# Autodesk Inventor assembly: Carcasa
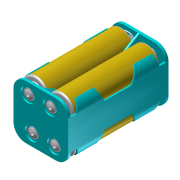
[picture p0: Inventor's stored thumbnail of the model, 180x180]
Saved by Autodesk Inventor 2013 (Build 170138000, 138)
## iProperties
Created: 2015-06-07
Part Number: Carcasa
Document SubType Name: Assembly
Designer: Luis
Author: Luis
## Documents named in this file (3)
- C:\Users\Luis\Documents\Inventor\Bateria\Carcasa.iam
- C:\Users\Luis\Documents\Inventor\Bateria\Imported Components\AABattery Holder\AABattery Holder.ipt
- C:\Users\Luis\Documents\Inventor\Bateria\Imported Components\battery-aa_1-5v\battery-aa_1-5v.ipt
## Components (6 placed, 2 different names)
1. AABattery Holder:1 — Mate:1, Flush:1, Flush:2, Tangent:1, Tangent:2, Mate:2, Tangent:3, Tangent:4, Mate:3
2. AABattery Holder:2 — Mate:1, Flush:1, Flush:2, Tangent:5, Tangent:6, Tangent:7, Tangent:8, Mate:4, Mate:5
3. battery-aa_1-5v:1 — Tangent:1, Tangent:2, Mate:2
4. battery-aa_1-5v:2 — Tangent:3, Tangent:4, Mate:3
5. battery-aa_1-5v:3 — Tangent:7, Tangent:8, Mate:4
6. battery-aa_1-5v:4 — Tangent:5, Tangent:6, Mate:5
## Relationships (15: Tangent 8, Mate 5, Flush 2)
- Mate:1 (-1 mm): AABattery Holder:1 ↔ AABattery Holder:2
- Flush:1: AABattery Holder:1 ↔ AABattery Holder:2
- Flush:2: AABattery Holder:1 ↔ AABattery Holder:2
- Tangent:1: AABattery Holder:1 ↔ battery-aa_1-5v:1
- Tangent:2: AABattery Holder:1 ↔ battery-aa_1-5v:1
- Mate:2 (2 mm): AABattery Holder:1 ↔ battery-aa_1-5v:1
- Tangent:3: AABattery Holder:1 ↔ battery-aa_1-5v:2
- Tangent:4: AABattery Holder:1 ↔ battery-aa_1-5v:2
- Mate:3 (2 mm): AABattery Holder:1 ↔ battery-aa_1-5v:2
- Tangent:5: AABattery Holder:2 ↔ battery-aa_1-5v:4
- Tangent:6: AABattery Holder:2 ↔ battery-aa_1-5v:4
- Tangent:7: AABattery Holder:2 ↔ battery-aa_1-5v:3
- Tangent:8: AABattery Holder:2 ↔ battery-aa_1-5v:3
- Mate:4 (2 mm): AABattery Holder:2 ↔ battery-aa_1-5v:3
- Mate:5 (2 mm): AABattery Holder:2 ↔ battery-aa_1-5v:4
